# Autodesk Inventor assembly: Schneckenräder
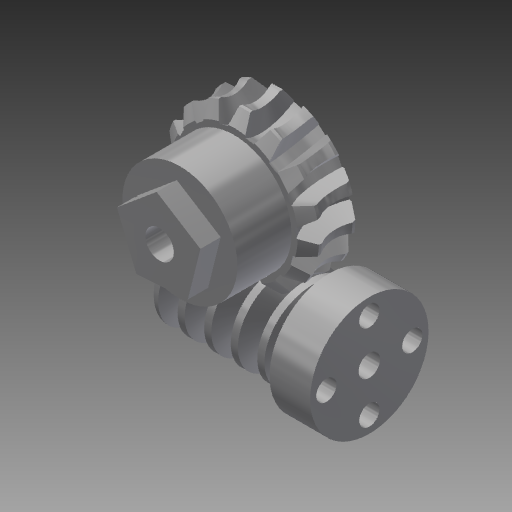
[picture p0: Inventor's stored thumbnail of the model, 512x512]
Saved by Autodesk Inventor 2019.1 (Build 231200000, 200)
## iProperties
Created: 2018-11-20
Part Number: Schneckenräder
Document SubType Name: Assembly
Designer: JochenAlt
Categories: <?xml version="1.0" encoding="UTF-16"?> <MemberInstance><Categories><FamilyTemplate/><ParamToTemplateMap><ParamToTemplate><ParamToTemplate CategoryParameter="//CategoryParameter[@InternalName='9E91F9C2-1A37-4abf-91CE-B4CF7EE75BC6']" ConstantValue="1000000.000000"/></ParamToTemplate><ParamToTemplate><ParamToTemplate CategoryParameter="//CategoryParameter[@InternalName='2AFF4D85-1BD8-4ea8-8D18-96A2CAB0895B']" ConstantValue="606612.952275"/></ParamToTemplate><ParamToTemplate><ParamToTemplate CategoryParameter="//CategoryParameter[@InternalName='E8E51088-10FD-40b5-B945-790B32C7EFBA']" ConstantValue="104.719755"/></ParamToTemplate><ParamToTemplate><ParamToTemplate CategoryParameter="//CategoryParameter[@InternalName='752D88A1-A866-440c-81C2-59259440B19C']" ConstantValue="6.981317"/></ParamToTemplate><ParamToTemplate><ParamToTemplate CategoryParameter="//CategoryParameter[@InternalName='5F43FD89-24D7-49f6-B63B-C3D8E39D8A69']" ConstantValue="9549.296586"/></ParamToTemplate><ParamToTemplate><ParamToTemplate CategoryParameter="//CategoryParameter[@InternalName='8D239626-6A17-497c-A9EF-C1C80B41D68F']" ConstantValue="86890.904908"/></ParamToTemplate><ParamToTemplate><ParamToTemplate CategoryParameter="//CategoryParameter[@InternalName='41D48E04-51D6-4192-AEE3-C42B8672B6EA']" ConstantValue="0.606613"/></ParamToTemplate><ParamToTemplate><ParamToTemplate CategoryParameter="//CategoryParameter[@InternalName='1E8174DF-B5EE-4822-A5FB-BCD9891126C3']" ConstantValue="9.000000"/></ParamToTemplate><ParamToTemplate><ParamToTemplate CategoryParameter="//CategoryParameter[@InternalName='20F5447C-47B1-4fb0-ACD5-EE92291F3ED6']" ConstantValue="0.390297"/></ParamToTemplate></ParamToTemplateMap><Category DisplayName="Gears" InternalName="3565AA18-AB10-415a-941E-C703DB507537" Mnemonic="Gears"><CategoryParameter DisplayName="P" InternalName="9E91F9C2-1A37-4abf-91CE-B4CF7EE75BC6" Mnemonic="P1"/><CategoryParameter DisplayName="P" InternalName="2AFF4D85-1BD8-4ea8-8D18-96A2CAB0895B" Mnemonic="P2"/><CategoryParameter DisplayName="n" InternalName="E8E51088-10FD-40b5-B945-790B32C7EFBA" Mnemonic="n1"/><CategoryParameter DisplayName="n" InternalName="752D88A1-A866-440c-81C2-59259440B19C" Mnemonic="n2"/><CategoryParameter DisplayName="T" InternalName="5F43FD89-24D7-49f6-B63B-C3D8E39D8A69" Mnemonic="Mk1"/><CategoryParameter DisplayName="T" InternalName="8D239626-6A17-497c-A9EF-C1C80B41D68F" Mnemonic="Mk2"/><CategoryParameter DisplayName="||h|" InternalName="41D48E04-51D6-4192-AEE3-C42B8672B6EA" Mnemonic="eta"/><Category DisplayName="WormGears" InternalName="2B10D032-4568-4ca1-81B6-0EE8891F8531" Mnemonic="WormGears"><CategoryParameter DisplayName="q" InternalName="1E8174DF-B5EE-4822-A5FB-BCD9891126C3" Mnemonic="q"/><CategoryParameter DisplayName="p|.n|" InternalName="20F5447C-47B1-4fb0-ACD5-EE92291F3ED6" Mnemonic="pn"/></Category></Category></Categories></MemberInstance>
ClientObjectVersion: 1
Author: JochenAlt
## Documents named in this file (3)
- D:\Projects\Ondine\CAD\Leg\Schnecke\Schneckenräder1.iam
- D:\Projects\Ondine\CAD\Leg\Schnecke\Schnecke1.ipt
- D:\Projects\Ondine\CAD\Leg\Schnecke\Schneckenrad1.ipt
## Components (2 placed, 2 different names)
1. Schnecke:1 — Passend:3, Drehung:1
2. Schneckenrad:1 — Passend:3, Drehung:1
## Relationships (3: Composite 1, Mate 1, RelateRotation 1)
- [Composite]: Schnecke:1 ↔ Schneckenrad:1
- Passend:3 [Mate] (15 mm): Schnecke:1 ↔ Schneckenrad:1
- Drehung:1 [RelateRotation] (0.0667 ul): Schnecke:1 ↔ Schneckenrad:1
